# Autodesk Inventor assembly: Assembly_motorcoverbase
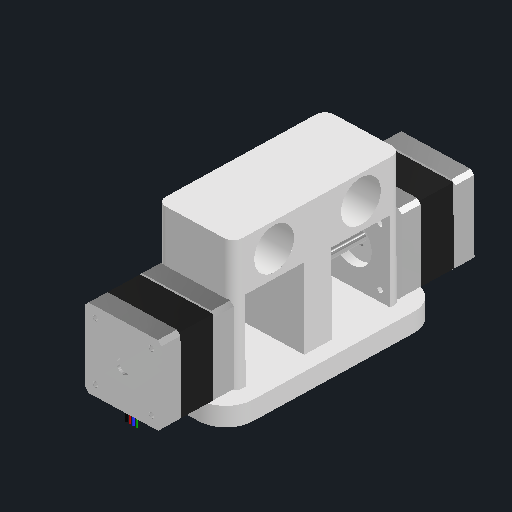
[picture p0: Inventor's stored thumbnail of the model, 512x512]
Saved by Autodesk Inventor 2024.2 (Build 282272000, 272)
## iProperties
Created: 2024-03-21
Part Number: Assembly_motorcoverbase
Document SubType Name: Assembly
Designer: seifs
Author: seifs
## Documents named in this file (8)
- C:\Users\seifs\Downloads\Final Assembly\Assembly_motorcoverbase.iam
- C:\Users\seifs\Downloads\Final Assembly\NEMA17 Stepper Motor.ipt
- C:\Users\seifs\Downloads\Final Assembly\LeadNut.ipt
- C:\Users\seifs\Downloads\Final Assembly\midle part.ipt
- C:\Users\seifs\Downloads\Final Assembly\ISO 7046-1 - M3 x 16_ - 4.8 - Z - ISO.ipt
- C:\Users\seifs\Downloads\Final Assembly\ISO 7046-1 - M3 x 20_ - 4.8 - Z - ISO.ipt
- C:\Users\seifs\Downloads\Final Assembly\ISO 4036 - M3(2).ipt
- C:\Users\seifs\Downloads\Final Assembly\NEMA17 Stepper Motor_MIR.ipt
## Components (16 placed, 7 different names)
1. LeadNut:1 — Insert:8, Insert:9, Insert:24, Insert:25, Insert:26, Insert:27
2. midle part:1 — Insert:8, Insert:9, Insert:20, Insert:21, Insert:22, Insert:23, Insert:32, Mate:2, Insert:33, Insert:34, Insert:35, Insert:36, Insert:37
3. ISO 7046-1 Z M3 x 20 - 4.8 - Z:1 — Insert:20
4. ISO 7046-1 Z M3 x 20 - 4.8 - Z:2 — Insert:21
5. ISO 7046-1 Z M3 x 20 - 4.8 - Z:3 — Insert:22
6. ISO 7046-1 Z M3 x 20 - 4.8 - Z:4 — Insert:23
7. ISO 4036 M3:1 — Insert:25
8. ISO 4036 M3:2 — Insert:27
9. ISO 4036 M3:3 — Insert:26
10. ISO 4036 M3:4 — Insert:24
11. NEMA17 Stepper Motor:2 — Insert:32, Mate:2
12. ISO 7046-1 Z M3 x 16 - 4.8 - Z:9 — Insert:35
13. ISO 7046-1 Z M3 x 16 - 4.8 - Z:10 — Insert:34
14. ISO 7046-1 Z M3 x 16 - 4.8 - Z:11 — Insert:36
15. ISO 7046-1 Z M3 x 16 - 4.8 - Z:12 — Insert:33
16. NEMA17 Stepper Motor_MIR:1 — Insert:37
## Relationships (17: Insert 16, Mate 1)
- Insert:8: LeadNut:1 ↔ midle part:1
- Insert:9: LeadNut:1 ↔ midle part:1
- Insert:20: midle part:1 ↔ ISO 7046-1 Z M3 x 20 - 4.8 - Z:1
- Insert:21: midle part:1 ↔ ISO 7046-1 Z M3 x 20 - 4.8 - Z:2
- Insert:22: midle part:1 ↔ ISO 7046-1 Z M3 x 20 - 4.8 - Z:3
- Insert:23: midle part:1 ↔ ISO 7046-1 Z M3 x 20 - 4.8 - Z:4
- Insert:24: LeadNut:1 ↔ ISO 4036 M3:4
- Insert:25: LeadNut:1 ↔ ISO 4036 M3:1
- Insert:26: LeadNut:1 ↔ ISO 4036 M3:3
- Insert:27: LeadNut:1 ↔ ISO 4036 M3:2
- Insert:32: midle part:1 ↔ NEMA17 Stepper Motor:2
- Mate:2: midle part:1 ↔ NEMA17 Stepper Motor:2
- Insert:33: midle part:1 ↔ ISO 7046-1 Z M3 x 16 - 4.8 - Z:12
- Insert:34: midle part:1 ↔ ISO 7046-1 Z M3 x 16 - 4.8 - Z:10
- Insert:35: midle part:1 ↔ ISO 7046-1 Z M3 x 16 - 4.8 - Z:9
- Insert:36: midle part:1 ↔ ISO 7046-1 Z M3 x 16 - 4.8 - Z:11
- Insert:37: midle part:1 ↔ NEMA17 Stepper Motor_MIR:1
